# Autodesk Inventor assembly: IOT-Trike
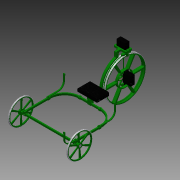
[picture p0: Inventor's stored thumbnail of the model, 180x180]
Saved by Autodesk Inventor 2014 SP1 (Build 180222100, 222)
## iProperties
Created: 2017-01-18
Part Number: IOT-Trike
Document SubType Name: Assembly
Designer: danielsikar
Author: danielsikar
## Documents named in this file (7)
- C:\Users\danielsikar\Documents\Inventor\IoT-Trike\Assemblies\IOT-Trike.iam
- C:\Users\danielsikar\Documents\Inventor\IoT-Trike\Assemblies\BackAxlePlusWheels.iam
- C:\Users\danielsikar\Documents\Inventor\IoT-Trike\Assemblies\ForkHandleBar.iam
- C:\Users\danielsikar\Documents\Inventor\IoT-Trike\Assemblies\Undercarriage.iam
- C:\Users\danielsikar\Documents\Inventor\IoT-Trike\Parts\MudGuard.ipt
- C:\Users\danielsikar\Documents\Inventor\IoT-Trike\Parts\MudGuardBrace.ipt
- C:\Users\danielsikar\Documents\Inventor\IoT-Trike\Parts\BatteryPack.ipt
## Components (6 placed, 6 different names)
1. BackAxlePlusWheels:1 [sub-assembly] — Flush:1, Mate:1, Mate:2, Mate:4, Mate:5, Mate:6
2. Undercarriage:1 [sub-assembly] — Mate:4, Mate:5, Mate:6, Mate:7, Flush:3, Mate:8, Mate:9
3. MudGuard:1 — Mate:7, Flush:3, Mate:8, Flush:4, Flush:5, Mate:10, Flush:6, Mate:11, Flush:7, Flush:8
4. MudGuardBrace:1 — Flush:4, Flush:5, Mate:9
5. BatteryPack:1 — Mate:10, Flush:6
6. ForkHandleBar:1 [sub-assembly] — Mate:11, Flush:7, Flush:8
## Relationships (17: Mate 10, Flush 7)
- Flush:1: BackAxlePlusWheels:1
- Mate:1: BackAxlePlusWheels:1
- Mate:2: BackAxlePlusWheels:1
- Mate:4: BackAxlePlusWheels:1 ↔ Undercarriage:1
- Mate:5: BackAxlePlusWheels:1 ↔ Undercarriage:1
- Mate:6: BackAxlePlusWheels:1 ↔ Undercarriage:1
- Mate:7: Undercarriage:1 ↔ MudGuard:1
- Flush:3: Undercarriage:1 ↔ MudGuard:1
- Mate:8: Undercarriage:1 ↔ MudGuard:1
- Flush:4: MudGuard:1 ↔ MudGuardBrace:1
- Flush:5: MudGuard:1 ↔ MudGuardBrace:1
- Mate:9: Undercarriage:1 ↔ MudGuardBrace:1
- Mate:10: MudGuard:1 ↔ BatteryPack:1
- Flush:6 (10 mm): MudGuard:1 ↔ BatteryPack:1
- Mate:11: MudGuard:1 ↔ ForkHandleBar:1
- Flush:7: MudGuard:1 ↔ ForkHandleBar:1
- Flush:8: MudGuard:1 ↔ ForkHandleBar:1
